# Autodesk Inventor assembly: hardpoint
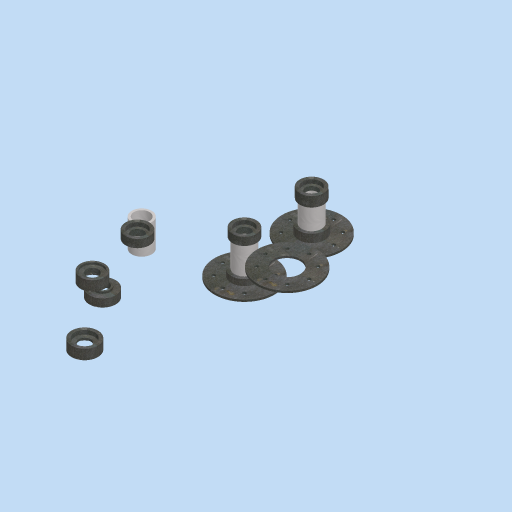
[picture p0: Inventor's stored thumbnail of the model, 512x512]
Saved by Autodesk Inventor 2023 (Build 270158000, 158)
## iProperties
Created: 2026-04-08
Part Number: hardpoint
Document SubType Name: Assembly
Designer: Nathann
Author: Nathann
## Documents named in this file (7)
- C:\Users\Nathann\ClawdDrive\Objet3D\neodrive\neodrive-cad-ergonomic-v1\eggshellCorePrinted\hardpoint.iam
- C:\Users\Nathann\ClawdDrive\Objet3D\neodrive\tube.ipt
- C:\Users\Nathann\ClawdDrive\Objet3D\neodrive\neodrive-cad-ergonomic-v1\eggshellCorePrinted\smallbearingcup.ipt
- C:\Users\Nathann\ClawdDrive\Objet3D\neodrive\neodrive-cad-ergonomic-v1\eggshellCorePrinted\bigbearingcup.ipt
- C:\Users\Nathann\ClawdDrive\Objet3D\neodrive\neodrive-cad-ergonomic-v1\eggshellCorePrinted\bigbearingcupInternalMachining.ipt
- C:\Users\Nathann\ClawdDrive\Objet3D\neodrive\neodrive-cad-ergonomic-v1\eggshellCorePrinted\smallbearingcupInternalMachining.ipt
- C:\Users\Nathann\ClawdDrive\Objet3D\neodrive\neodrive-cad-ergonomic-v1\eggshellCorePrinted\plateHole.ipt
## Components (14 placed, 6 different names)
1. tube:1 — Insert:1, Insert:2
2. smallbearingcup:1 — Insert:1
3. bigbearingcup:1
4. smallbearingcup:2
5. bigbearingcup:2 — Insert:2, Insert:5
6. tube:2
7. bigbearingcupInternalMachining:1
8. smallbearingcupInternalMachining:1
9. tube:3 — Insert:3, Insert:4
10. bigbearingcupInternalMachining:2 — Insert:4, Insert:6
11. smallbearingcupInternalMachining:2 — Insert:3
12. plateHole:1 — Insert:6
13. plateHole:2
14. plateHole:4 — Insert:5
## Relationships (6: Insert 6)
- Insert:1: tube:1 ↔ smallbearingcup:1
- Insert:2: tube:1 ↔ bigbearingcup:2
- Insert:3: tube:3 ↔ smallbearingcupInternalMachining:2
- Insert:4: tube:3 ↔ bigbearingcupInternalMachining:2
- Insert:5 (-5 mm): bigbearingcup:2 ↔ plateHole:4
- Insert:6 (-5 mm): bigbearingcupInternalMachining:2 ↔ plateHole:1
